# Autodesk Inventor assembly: Fixation_CPY
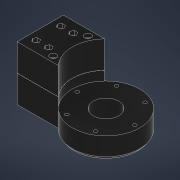
[picture p0: Inventor's stored thumbnail of the model, 180x180]
Saved by Autodesk Inventor 2021 (Build 250183000, 183)
## iProperties
Created: 2025-04-02
Part Number: Fixation_CPY
Document SubType Name: Assembly
Designer: rocke
Author: rocke
## Documents named in this file (3)
- C:\Users\rocke\Documents\Robot Arm IPT\Fixation_CPY.iam
- C:\Users\rocke\Documents\Robot Arm IPT\Left_CPY.ipt
- C:\Users\rocke\Documents\Robot Arm IPT\Left_CPY_CPY.ipt
## Components (2 placed, 2 different names)
1. Left_CPY:1 — Insert:1
2. Left_CPY_CPY:1 — Insert:1
## Relationships (1: Insert 1)
- Insert:1: Left_CPY:1 ↔ Left_CPY_CPY:1
